# Autodesk Inventor assembly: CJ2B16-100Z
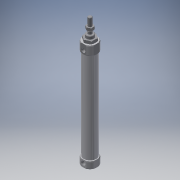
[picture p0: Inventor's stored thumbnail of the model, 180x180]
Saved by Autodesk Inventor 2017 (Build 210142000, 142)
## iProperties
Created: 2017-12-08
Part Number: CJ2B16-100Z
Document SubType Name: Assembly
Designer: RLanting
Sending System: SolidWorks 2017
Major Version: 7.0
Minor Version: 0.0
Format Version: 0.0
Product Id: SolidWorks 2017
Author: RLanting
## Documents named in this file (7)
- E:\direct drive electronic valving 2\hydraulic steering\CJ2B16-100Z.iam
- E:\direct drive electronic valving 2\hydraulic steering\CJ2B16-100Z.ipt
- E:\direct drive electronic valving 2\hydraulic steering\CJ2B16-100Z_1.ipt
- E:\direct drive electronic valving 2\hydraulic steering\CJ2B16-100Z_2.ipt
- E:\direct drive electronic valving 2\hydraulic steering\CJ2B16-100Z_3.ipt
- E:\direct drive electronic valving 2\hydraulic steering\CJ2B16-100Z_4.ipt
- E:\direct drive electronic valving 2\hydraulic steering\CJ2B16-100Z_5.ipt
## Components (6 placed, 6 different names)
1. CJ2B16-100Z_1:1 — Mate:1, Mate:2, Mate:3, Mate:4, Mate:5
2. CJ2B16-100Z_2:1 — Mate:3, Mate:4, Angle:1, Mate:6, Mate:7, Flush:2
3. CJ2B16-100Z_3:1 — Mate:1, Mate:2, Angle:1, Angle:2
4. CJ2B16-100Z_4:1 — Mate:5, Flush:1, Mate:8, Flush:2
5. CJ2B16-100Z_5:1 — Mate:6, Mate:7
6. CJ2B16-100Z_6:1 — Flush:1, Mate:8
## Relationships (12: Mate 8, Angle 2, Flush 2)
- Mate:1: CJ2B16-100Z_1:1 ↔ CJ2B16-100Z_3:1
- Mate:2: CJ2B16-100Z_1:1 ↔ CJ2B16-100Z_3:1
- Mate:3: CJ2B16-100Z_1:1 ↔ CJ2B16-100Z_2:1
- Mate:4: CJ2B16-100Z_1:1 ↔ CJ2B16-100Z_2:1
- Angle:1 (0 deg): CJ2B16-100Z_2:1 ↔ CJ2B16-100Z_3:1
- Angle:2 (0 deg): CJ2B16-100Z_3:1
- Mate:5: CJ2B16-100Z_1:1 ↔ CJ2B16-100Z_4:1
- Mate:6: CJ2B16-100Z_2:1 ↔ CJ2B16-100Z_5:1
- Mate:7: CJ2B16-100Z_2:1 ↔ CJ2B16-100Z_5:1
- Flush:1: CJ2B16-100Z_4:1 ↔ CJ2B16-100Z_6:1
- Mate:8: CJ2B16-100Z_4:1 ↔ CJ2B16-100Z_6:1
- Flush:2 (-28 mm): CJ2B16-100Z_2:1 ↔ CJ2B16-100Z_4:1
